# Autodesk Inventor assembly: 000.012 - Крепление XT60 папа
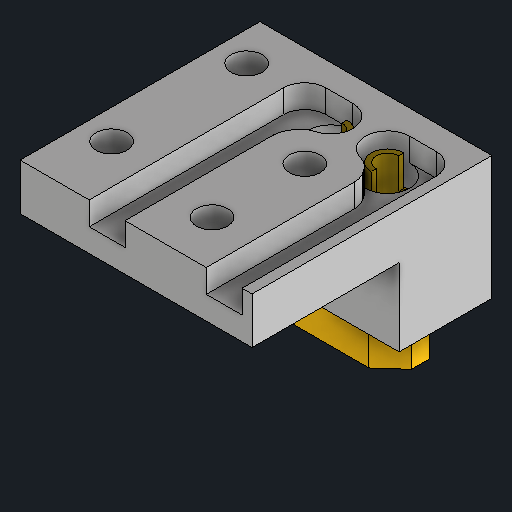
[picture p0: Inventor's stored thumbnail of the model, 512x512]
Saved by Autodesk Inventor 2025 (Build 290162000, 162)
## iProperties
Created: 2023-04-23
Part Number: 000.012 - Крепление XT60 папа
Document SubType Name: Assembly
Designer: Иван Петров
Author: Иван Петров
## Documents named in this file (3)
- D:\Projects\OmniBot\design\000.004 - Крепление XT60 папа.iam
- D:\Projects\OmniBot\design\000.004.001 - Основание.ipt
- D:\Projects\OmniBot\design\standart_components\XT60FemaleConnector.ipt
## Components (2 placed, 2 different names)
1. 000.004.001 - Основание:1 — Совмещение:1
2. XT60FemaleConnector:1 — Совмещение:1
## Relationships (1: Mate 1)
- Совмещение:1 [Mate]: 000.004.001 - Основание:1 ↔ XT60FemaleConnector:1
